# Autodesk Inventor assembly: Bolt_With_Washer
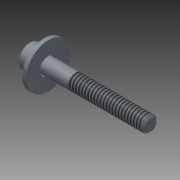
[picture p0: Inventor's stored thumbnail of the model, 180x180]
Saved by Autodesk Inventor 2013 (Build 170138000, 138)
## iProperties
Created: 2013-07-13
Part Number: Bolt_With_Washer
Document SubType Name: Assembly
Designer: orange
Author: orange
## Documents named in this file (3)
- H:\Inventor_Projects\Shooter_No_Welding\Base\Bolt_With_Washer.iam
- H:\Inventor_Projects\Shooter_No_Welding\UnmoddedKOP\DBK_14-20x175_SHCS_am-1058.ipt
- H:\Inventor_Projects\Shooter_No_Welding\UnmoddedKOP\DBK_14Washer_am-1027.ipt
## Components (2 placed, 2 different names)
1. DBK_14-20x175_SHCS_am-1058:1 — Mate:1, Mate:2
2. DBK_14Washer_am-1027:1 — Mate:1, Mate:2
## Relationships (2: Mate 2)
- Mate:1: DBK_14-20x175_SHCS_am-1058:1 ↔ DBK_14Washer_am-1027:1
- Mate:2: DBK_14-20x175_SHCS_am-1058:1 ↔ DBK_14Washer_am-1027:1
